# Autodesk Inventor assembly: robot
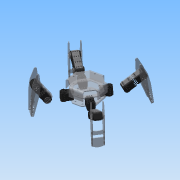
[picture p0: Inventor's stored thumbnail of the model, 180x180]
Saved by Autodesk Inventor 2015 (Build 190159000, 159)
## iProperties
Created: 2016-03-01
Part Number: robot
Document SubType Name: Assembly
Designer: Gregwar
Author: Gregwar
## Documents named in this file (10)
- C:\Users\Gregwar\Desktop\Metabot\mechanics\laser\autodesk\robot.iam
- C:\Users\Gregwar\Desktop\Metabot\mechanics\laser\autodesk\models\motor_arm.iam
- C:\Users\Gregwar\Desktop\Metabot\mechanics\laser\autodesk\u.ipt
- C:\Users\Gregwar\Desktop\Metabot\mechanics\laser\autodesk\side.ipt
- C:\Users\Gregwar\Desktop\Metabot\mechanics\laser\autodesk\leg.ipt
- C:\Users\Gregwar\Desktop\Metabot\mechanics\laser\autodesk\tip.ipt
- C:\Users\Gregwar\Desktop\Metabot\mechanics\laser\autodesk\tip_up.ipt
- C:\Users\Gregwar\Desktop\Metabot\mechanics\laser\autodesk\body_bottom.ipt
- C:\Users\Gregwar\Desktop\Metabot\mechanics\laser\autodesk\body_top.ipt
- C:\Users\Gregwar\Desktop\Metabot\mechanics\laser\autodesk\head.ipt
## Components (43 placed, 9 different names)
1. motor_arm:1 [sub-assembly] — Placage:1, Placage:2, Placage:25, Placage:26, Placage:27, Placage:28, Placage:29, Placage:30
2. u:1 — Placage:1, Placage:2, Placage:3, Placage:4, Placage:5
3. u:2 — Placage:3, Placage:4, Placage:5, Placage:6, Placage:7
4. motor_arm:2 [sub-assembly] — Placage:6, Placage:7, Placage:8, Placage:9, Placage:10
5. side:1 — Placage:8, Placage:9, Placage:10, Placage:11, Placage:12, Placage:13
6. motor_arm:3 [sub-assembly] — Placage:11, Placage:12, Placage:13, Placage:14, Placage:15, Placage:16, Placage:17
7. leg:1 — Placage:14, Placage:15, Placage:20, Placage:21, Placage:22, Placage:23, Placage:24
8. leg:2 — Placage:16, Placage:17, Placage:18, Placage:19
9. tip:1 — Placage:18, Placage:19, Placage:20, Placage:24
10. tip_up:1 — Placage:21, Placage:22, Placage:23
11. body_bottom:1 — Placage:25, Placage:26, Placage:27, Placage:60, Placage:61, Placage:62, Placage:87, Placage:88, Placage:89, Placage:114, Placage:115, Placage:116
12. body_top:1 — Placage:28, Placage:29, Placage:30, Placage:117, Placage:118, Placage:119
13. motor_arm:4 [sub-assembly] — Placage:60, Placage:61, Placage:62
14. u:3
15. u:4
16. motor_arm:5 [sub-assembly]
17. side:2
18. motor_arm:6 [sub-assembly]
19. leg:3
20. leg:4
21. tip:2
22. tip_up:2
23. motor_arm:7 [sub-assembly] — Placage:87, Placage:88, Placage:89
24. u:5
25. u:6
26. motor_arm:8 [sub-assembly]
27. side:3
28. motor_arm:9 [sub-assembly]
29. leg:5
30. leg:6
31. tip:3
32. tip_up:3
33. motor_arm:10 [sub-assembly] — Placage:114, Placage:115, Placage:116
34. u:7
35. u:8
36. motor_arm:11 [sub-assembly]
37. side:4
38. motor_arm:12 [sub-assembly]
39. leg:7
40. leg:8
41. tip:4
42. tip_up:4
43. head:1 — Placage:117, Placage:118, Placage:119
## Relationships (114: Mate 114)
- Placage:1 [Mate]: motor_arm:1 ↔ u:1
- Placage:2 [Mate]: motor_arm:1 ↔ u:1
- Placage:3 [Mate]: u:1 ↔ u:2
- Placage:4 [Mate]: u:1 ↔ u:2
- Placage:5 [Mate]: u:1 ↔ u:2
- Placage:6 [Mate]: u:2 ↔ motor_arm:2
- Placage:7 [Mate]: u:2 ↔ motor_arm:2
- Placage:8 [Mate]: motor_arm:2 ↔ side:1
- Placage:9 [Mate]: motor_arm:2 ↔ side:1
- Placage:10 [Mate]: motor_arm:2 ↔ side:1
- Placage:11 [Mate]: side:1 ↔ motor_arm:3
- Placage:12 [Mate]: side:1 ↔ motor_arm:3
- Placage:13 [Mate]: side:1 ↔ motor_arm:3
- Placage:14 [Mate]: motor_arm:3 ↔ leg:1
- Placage:15 [Mate]: motor_arm:3 ↔ leg:1
- Placage:16 [Mate]: motor_arm:3 ↔ leg:2
- Placage:17 [Mate]: motor_arm:3 ↔ leg:2
- Placage:18 [Mate]: leg:2 ↔ tip:1
- Placage:19 [Mate]: leg:2 ↔ tip:1
- Placage:20 [Mate]: leg:1 ↔ tip:1
- Placage:21 [Mate]: leg:1 ↔ tip_up:1
- Placage:22 [Mate]: leg:1 ↔ tip_up:1
- Placage:23 [Mate]: leg:1 ↔ tip_up:1
- Placage:24 [Mate]: leg:1 ↔ tip:1
- Placage:25 [Mate]: motor_arm:1 ↔ body_bottom:1
- Placage:26 [Mate]: motor_arm:1 ↔ body_bottom:1
- Placage:27 [Mate]: motor_arm:1 ↔ body_bottom:1
- Placage:28 [Mate]: motor_arm:1 ↔ body_top:1
- Placage:29 [Mate]: motor_arm:1 ↔ body_top:1
- Placage:30 [Mate]: motor_arm:1 ↔ body_top:1
- [Mate]: motor_arm:4 ↔ u:3
- [Mate]: motor_arm:4 ↔ u:3
- [Mate]: u:3 ↔ u:4
- [Mate]: u:3 ↔ u:4
- [Mate]: u:3 ↔ u:4
- [Mate]: u:4 ↔ motor_arm:5
- [Mate]: u:4 ↔ motor_arm:5
- [Mate]: motor_arm:5 ↔ side:2
- [Mate]: motor_arm:5 ↔ side:2
- [Mate]: motor_arm:5 ↔ side:2
- [Mate]: side:2 ↔ motor_arm:6
- [Mate]: side:2 ↔ motor_arm:6
- [Mate]: side:2 ↔ motor_arm:6
- [Mate]: motor_arm:6 ↔ leg:3
- [Mate]: motor_arm:6 ↔ leg:3
- [Mate]: motor_arm:6 ↔ leg:4
- [Mate]: motor_arm:6 ↔ leg:4
- [Mate]: leg:4 ↔ tip:2
- [Mate]: leg:4 ↔ tip:2
- [Mate]: leg:3 ↔ tip:2
- [Mate]: leg:3 ↔ tip_up:2
- [Mate]: leg:3 ↔ tip_up:2
- [Mate]: leg:3 ↔ tip_up:2
- [Mate]: leg:3 ↔ tip:2
- Placage:60 [Mate]: body_bottom:1 ↔ motor_arm:4
- Placage:61 [Mate]: body_bottom:1 ↔ motor_arm:4
- Placage:62 [Mate]: body_bottom:1 ↔ motor_arm:4
- [Mate]: motor_arm:7 ↔ u:5
- [Mate]: motor_arm:7 ↔ u:5
- [Mate]: u:5 ↔ u:6
- [Mate]: u:5 ↔ u:6
- [Mate]: u:5 ↔ u:6
- [Mate]: u:6 ↔ motor_arm:8
- [Mate]: u:6 ↔ motor_arm:8
- [Mate]: motor_arm:8 ↔ side:3
- [Mate]: motor_arm:8 ↔ side:3
- [Mate]: motor_arm:8 ↔ side:3
- [Mate]: side:3 ↔ motor_arm:9
- [Mate]: side:3 ↔ motor_arm:9
- [Mate]: side:3 ↔ motor_arm:9
- [Mate]: motor_arm:9 ↔ leg:5
- [Mate]: motor_arm:9 ↔ leg:5
- [Mate]: motor_arm:9 ↔ leg:6
- [Mate]: motor_arm:9 ↔ leg:6
- [Mate]: leg:6 ↔ tip:3
- [Mate]: leg:6 ↔ tip:3
- [Mate]: leg:5 ↔ tip:3
- [Mate]: leg:5 ↔ tip_up:3
- [Mate]: leg:5 ↔ tip_up:3
- [Mate]: leg:5 ↔ tip_up:3
- [Mate]: leg:5 ↔ tip:3
- Placage:87 [Mate]: body_bottom:1 ↔ motor_arm:7
- Placage:88 [Mate]: body_bottom:1 ↔ motor_arm:7
- Placage:89 [Mate]: body_bottom:1 ↔ motor_arm:7
- [Mate]: motor_arm:10 ↔ u:7
- [Mate]: motor_arm:10 ↔ u:7
- [Mate]: u:7 ↔ u:8
- [Mate]: u:7 ↔ u:8
- [Mate]: u:7 ↔ u:8
- [Mate]: u:8 ↔ motor_arm:11
- [Mate]: u:8 ↔ motor_arm:11
- [Mate]: motor_arm:11 ↔ side:4
- [Mate]: motor_arm:11 ↔ side:4
- [Mate]: motor_arm:11 ↔ side:4
- [Mate]: side:4 ↔ motor_arm:12
- [Mate]: side:4 ↔ motor_arm:12
- [Mate]: side:4 ↔ motor_arm:12
- [Mate]: motor_arm:12 ↔ leg:7
- [Mate]: motor_arm:12 ↔ leg:7
- [Mate]: motor_arm:12 ↔ leg:8
- [Mate]: motor_arm:12 ↔ leg:8
- [Mate]: leg:8 ↔ tip:4
- [Mate]: leg:8 ↔ tip:4
- [Mate]: leg:7 ↔ tip:4
- [Mate]: leg:7 ↔ tip_up:4
- [Mate]: leg:7 ↔ tip_up:4
- [Mate]: leg:7 ↔ tip_up:4
- [Mate]: leg:7 ↔ tip:4
- Placage:114 [Mate]: body_bottom:1 ↔ motor_arm:10
- Placage:115 [Mate]: body_bottom:1 ↔ motor_arm:10
- Placage:116 [Mate]: body_bottom:1 ↔ motor_arm:10
- Placage:117 [Mate] (20 mm): body_top:1 ↔ head:1
- Placage:118 [Mate]: body_top:1 ↔ head:1
- Placage:119 [Mate]: body_top:1 ↔ head:1
## Named parameters: d41_d3 = 0 mm, d42_d4 = 0 mm, d43_d5 = 0 mm, d44_d6 = 0 mm, d45_d7 = 0 mm, d46_d8 = 0 mm, d47_d9 = 0 mm, d48_d10 = 0 mm, d49_d11 = 0 mm, d50_d12 = 0 mm, d51_d13 = 0 mm, d52_d14 = 0 mm, d53_d15 = 0 mm, d54_d16 = 0 mm, d55_d17 = 0 mm, d56_d0 = 0 mm, d57_d1 = 0 mm, d58_d2 = 0 mm, d59_d18 = 0 mm, d60_d19 = 0 mm, d61_d20 = 0 mm, d62_d21 = 0 mm, d63_d22 = 0 mm, d64_d23 = 0 mm, d68_d3 = 0 mm, d69_d4 = 0 mm, d70_d5 = 0 mm, d71_d6 = 0 mm, d72_d7 = 0 mm, d73_d8 = 0 mm, d74_d9 = 0 mm, d75_d10 = 0 mm, d76_d11 = 0 mm, d77_d12 = 0 mm, d78_d13 = 0 mm, d79_d14 = 0 mm, d80_d15 = 0 mm, d81_d16 = 0 mm, d82_d17 = 0 mm, d83_d0 = 0 mm, d84_d1 = 0 mm, d85_d2 = 0 mm, d86_d18 = 0 mm, d87_d19 = 0 mm, d88_d20 = 0 mm, d89_d21 = 0 mm, d90_d22 = 0 mm, d91_d23 = 0 mm, d95_d3 = 0 mm, d96_d4 = 0 mm, d97_d5 = 0 mm, d98_d6 = 0 mm, d99_d7 = 0 mm, d100_d8 = 0 mm, d101_d9 = 0 mm, d102_d10 = 0 mm, d103_d11 = 0 mm, d104_d12 = 0 mm, d105_d13 = 0 mm, d106_d14 = 0 mm, d107_d15 = 0 mm, d108_d16 = 0 mm, d109_d17 = 0 mm, d110_d0 = 0 mm, d111_d1 = 0 mm, d112_d2 = 0 mm, d113_d18 = 0 mm, d114_d19 = 0 mm, d115_d20 = 0 mm, d116_d21 = 0 mm, d117_d22 = 0 mm, d118_d23 = 0 mm
